# Autodesk Inventor assembly: lustro_i_dmd
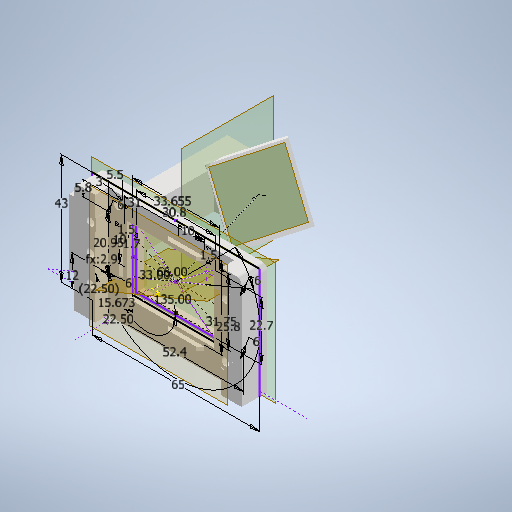
[picture p0: Inventor's stored thumbnail of the model, 512x512]
Saved by Autodesk Inventor 2025.1 (Build 291241020, 241B)
## iProperties
Created: 2024-10-13
Part Number: lustro_i_dmd
Document SubType Name: Assembly
Designer: zychlix
Author: zychlix
## Documents named in this file (4)
- C:\Users\zychlix\Fotolitografia\lustro_i_dmd.iam
- C:\Users\zychlix\Fotolitografia\clamp.ipt
- C:\Users\zychlix\Fotolitografia\Część10.ipt
- C:\Users\zychlix\Fotolitografia\uchwycik_lustra.ipt
## Components (3 placed, 3 different names)
1. clamp:1 — Równoległe:1, Równoległe:2, Zestawiające:2, Zestawiające:3, Równoległe:3, Zestawiające:4, Równoległe:6
2. Część10:1 — Równoległe:1, Równoległe:2, Zestawiające:2, Zestawiające:3, Równoległe:4, Równoległe:5
3. uchwycik_lustra:1 — Równoległe:3, Równoległe:4, Równoległe:5, Zestawiające:4, Równoległe:6
## Relationships (9: Flush 6, Mate 3)
- Równoległe:1 [Flush]: clamp:1 ↔ Część10:1
- Równoległe:2 [Flush] (5 mm): clamp:1 ↔ Część10:1
- Zestawiające:2 [Mate]: clamp:1 ↔ Część10:1
- Zestawiające:3 [Mate]: clamp:1 ↔ Część10:1
- Równoległe:3 [Flush]: clamp:1 ↔ uchwycik_lustra:1
- Równoległe:4 [Flush]: Część10:1 ↔ uchwycik_lustra:1
- Równoległe:5 [Flush]: Część10:1 ↔ uchwycik_lustra:1
- Zestawiające:4 [Mate]: clamp:1 ↔ uchwycik_lustra:1
- Równoległe:6 [Flush]: clamp:1 ↔ uchwycik_lustra:1
